# Autodesk Inventor assembly: RR_SingleTurnout-BwoS
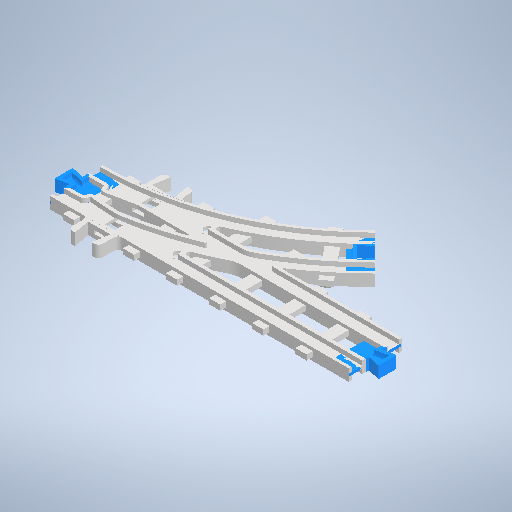
[picture p0: Inventor's stored thumbnail of the model, 512x512]
Saved by Autodesk Inventor 2025.1 (Build 291241000, 241)
## iProperties
Created: 2025-03-06
Part Number: RR_SingleTurnout-BwoS
Document SubType Name: Assembly
Designer: kumagai
Author: kumagai
## Documents named in this file (11)
- X:\Develop\CAD\PlaRails\RealRails\RR_SingleTurnout.iam
- X:\Develop\CAD\PlaRails\RealRails\RR_SingleTurnout.ipt
- X:\Develop\CAD\PlaRails\Common\RailJointRS.ipt
- X:\Develop\CAD\PlaRails\RealRails\RR_SingleTurnout_Pillow.ipt
- X:\Develop\CAD\PlaRails\RealRails\RR_SingleTurnout\RR_SingleTurnout-railcon.ipt
- X:\Develop\CAD\PlaRails\Common\RailJointRS\FemaleDoubleSide.ipt
- X:\Develop\CAD\PlaRails\Common\RailJointRS\MaleDoubleSide.ipt
- RR_SingleTurnout-A.iam
- RR_SingleTurnout-AwoS.iam
- RR_SingleTurnout-B.iam
- RR_SingleTurnout-BwoS.iam
## Components (5 placed, 4 different names)
1. RR_SingleTurnout-railcon:1 — フラッシュ:1, メイト:1, フラッシュ:2, フラッシュ:3, メイト:2, フラッシュ:4, フラッシュ:5, メイト:3, フラッシュ:6
2. MaleDoubleSide:1 — フラッシュ:1, メイト:1, フラッシュ:2
3. MaleDoubleSide:2 — フラッシュ:3, メイト:2, フラッシュ:4
4. FemaleDoubleSide:3 — フラッシュ:5, メイト:3, フラッシュ:6
5. RR_SingleTurnout_Pillow:1
## Relationships (9: Flush 6, Mate 3)
- フラッシュ:1 [Flush]: RR_SingleTurnout-railcon:1 ↔ MaleDoubleSide:1
- メイト:1 [Mate]: RR_SingleTurnout-railcon:1 ↔ MaleDoubleSide:1
- フラッシュ:2 [Flush]: RR_SingleTurnout-railcon:1 ↔ MaleDoubleSide:1
- フラッシュ:3 [Flush]: RR_SingleTurnout-railcon:1 ↔ MaleDoubleSide:2
- メイト:2 [Mate]: RR_SingleTurnout-railcon:1 ↔ MaleDoubleSide:2
- フラッシュ:4 [Flush]: RR_SingleTurnout-railcon:1 ↔ MaleDoubleSide:2
- フラッシュ:5 [Flush]: RR_SingleTurnout-railcon:1 ↔ FemaleDoubleSide:3
- メイト:3 [Mate]: RR_SingleTurnout-railcon:1 ↔ FemaleDoubleSide:3
- フラッシュ:6 [Flush]: RR_SingleTurnout-railcon:1 ↔ FemaleDoubleSide:3
